# Autodesk Inventor assembly: ServoShaftCouplerAssembly
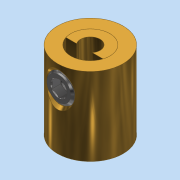
[picture p0: Inventor's stored thumbnail of the model, 180x180]
Saved by Autodesk Inventor 2017 (Build 210142000, 142)
## iProperties
Created: 2017-11-01
Part Number: ServoShaftCouplerAssembly
Document SubType Name: Assembly
Designer: Derek Wider
Author: Derek Wider
## Documents named in this file (4)
- G:\Projects\Submarine\Submarine-project\CAD\midships\AftServoSection\ServoShaftCoupler\ServoShaftCouplerAssembly.iam
- G:\Projects\Submarine\Submarine-project\CAD\midships\AftServoSection\ServoShaftCoupler\ShaftCoupler.ipt
- G:\Projects\Submarine\Submarine-project\CAD\midships\AftServoSection\ServoShaftCoupler\ShaftCollar.ipt
- G:\Projects\Submarine\Submarine-project\CAD\midships\AftServoSection\ServoShaftCoupler\SetScrew.ipt
## Components (3 placed, 3 different names)
1. ShaftCoupler:1 — Mate:2, Mate:3, Mate:4
2. ShaftCollar:1 — Mate:2, Mate:3, Flush:1
3. SetScrew:1 — Mate:4, Flush:1
## Relationships (4: Mate 3, Flush 1)
- Mate:2: ShaftCoupler:1 ↔ ShaftCollar:1
- Mate:3: ShaftCoupler:1 ↔ ShaftCollar:1
- Mate:4: ShaftCoupler:1 ↔ SetScrew:1
- Flush:1 (-4.191 mm): ShaftCollar:1 ↔ SetScrew:1
